# Autodesk Inventor assembly: EL2-GB-200
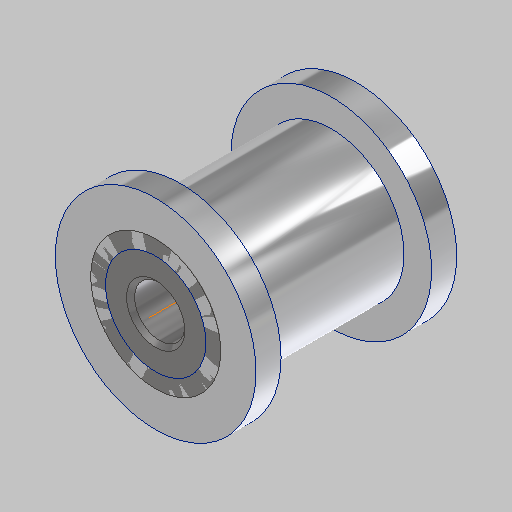
[picture p0: Inventor's stored thumbnail of the model, 512x512]
Saved by Autodesk Inventor 2023.5 (Build 275446000, 446)
## iProperties
Created: 2025-01-11
Part Number: EL2-GB-200
Document SubType Name: Assembly
Designer: mavericks
Author: mavericks
## Documents named in this file (3)
- C:\Users\slick\OneDrive\Desktop\2025-ReefScape---CAD\Elevator\EL2-GB\EL2-GB-200.iam
- C:\Users\slick\OneDrive\Desktop\2025-ReefScape---CAD\Elevator\EL2\EL2-007.ipt
- C:\Users\slick\OneDrive\Desktop\2025-ReefScape---CAD\COMMON PARTS\BEARINGS\Ball Bearing 1_4x11_16x5_16 Sealed 1602DC 1602-2RS.ipt
## Components (3 placed, 2 different names)
1. EL2-007:1 — Mate:1, Mate:2, Flush:1, Flush:2
2. Ball Bearing 1_4x11_16x5_16 Sealed 1602DC 1602-2RS:1 — Mate:2, Flush:1
3. Ball Bearing 1_4x11_16x5_16 Sealed 1602DC 1602-2RS:2 — Mate:1, Flush:2
## Relationships (4: Mate 2, Flush 2)
- Mate:1: EL2-007:1 ↔ Ball Bearing 1_4x11_16x5_16 Sealed 1602DC 1602-2RS:2
- Mate:2: EL2-007:1 ↔ Ball Bearing 1_4x11_16x5_16 Sealed 1602DC 1602-2RS:1
- Flush:1: EL2-007:1 ↔ Ball Bearing 1_4x11_16x5_16 Sealed 1602DC 1602-2RS:1
- Flush:2: EL2-007:1 ↔ Ball Bearing 1_4x11_16x5_16 Sealed 1602DC 1602-2RS:2
